# Autodesk Inventor assembly: Ball Screw Long
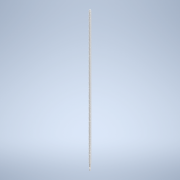
[picture p0: Inventor's stored thumbnail of the model, 180x180]
Saved by Autodesk Inventor 2022.3 (Build 263350000, 350)
## iProperties
Created: 2022-06-11
Part Number: Ball Screw Long
Document SubType Name: Assembly
Designer: Robert Nies
Author: Robert Nies
## Documents named in this file (4)
- C:\Users\rober\PycharmProjects\CNCRouter\Stock Parts\Linear Motion\Ball Screw Long.iam
- C:\Users\rober\PycharmProjects\CNCRouter\Stock Parts\Linear Motion\Ball Screw Middle.ipt
- C:\Users\rober\PycharmProjects\CNCRouter\Stock Parts\Linear Motion\Ball Screw Bottom.ipt
- C:\Users\rober\PycharmProjects\CNCRouter\Stock Parts\Linear Motion\Ball Screw Top.ipt
## Components (10 placed, 3 different names)
1. Ball Screw Middle:1 — Rigid:1, Rigid:9
2. Ball Screw Middle:2 — Rigid:1, Rigid:3
3. Ball Screw Middle:3 — Rigid:7
4. Ball Screw Middle:4 — Rigid:3
5. Ball Screw Middle:5 — Rigid:8
6. Ball Screw Middle:6
7. Ball Screw Middle:7 — Rigid:7
8. Ball Screw Middle:8
9. Ball Screw Bottom:1 — Rigid:9
10. Ball Screw Top:1 — Rigid:8
## Relationships (9: WeldJoint 9)
- Rigid:1 [WeldJoint]: Ball Screw Middle:1 ↔ Ball Screw Middle:2
- [WeldJoint]: Ball Screw Middle:3 ↔ Ball Screw Middle:4
- Rigid:3 [WeldJoint]: Ball Screw Middle:2 ↔ Ball Screw Middle:4
- [WeldJoint]: Ball Screw Middle:5 ↔ Ball Screw Middle:6
- [WeldJoint]: Ball Screw Middle:7 ↔ Ball Screw Middle:8
- [WeldJoint]: Ball Screw Middle:6 ↔ Ball Screw Middle:8
- Rigid:7 [WeldJoint]: Ball Screw Middle:3 ↔ Ball Screw Middle:7
- Rigid:8 [WeldJoint]: Ball Screw Middle:5 ↔ Ball Screw Top:1
- Rigid:9 [WeldJoint]: Ball Screw Middle:1 ↔ Ball Screw Bottom:1
## Named parameters: d1_d0 = 0 mm, d4_d0 = 0 mm, d5_d1_d0 = 0 mm, d6_d3 = 0 mm
